# Autodesk Inventor assembly: Core
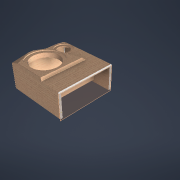
[picture p0: Inventor's stored thumbnail of the model, 180x180]
Saved by Autodesk Inventor 2022 (Build 260153000, 153)
## iProperties
Created: 2022-04-08
Part Number: Core
Document SubType Name: Assembly
Designer: Kalugin_a
Author: Kalugin_a
## Documents named in this file (9)
- D:\GitHUB\MELAS\Workspace\BoordyaBeatBox\Core.iam
- D:\GitHUB\MELAS\Workspace\BoordyaBeatBox\Front_L.ipt
- D:\GitHUB\MELAS\Workspace\BoordyaBeatBox\Front1.ipt
- Front1-hover.ipt
- D:\GitHUB\MELAS\Workspace\BoordyaBeatBox\Top.ipt
- D:\GitHUB\MELAS\Workspace\BoordyaBeatBox\side.ipt
- D:\GitHUB\MELAS\Workspace\BoordyaBeatBox\bottom.ipt
- D:\GitHUB\MELAS\Workspace\DIII\внутр.ipt
- D:\GitHUB\MELAS\Workspace\DIII\задник.ipt
## Components (8 placed, 7 different names)
1. Front_L:1 — Совмещение:1, Совмещение:2
2. Front1-hover:1
3. Top:1 — Совмещение:2, Совмещение:3, Совмещение:4
4. side:1 — Совмещение:1, Совмещение:3, Совмещение:5
5. bottom:1
6. side:2
7. внутр:1
8. задник:1 — Совмещение:4, Совмещение:5
## Relationships (5: Mate 5)
- Совмещение:1 [Mate]: Front_L:1 ↔ side:1
- Совмещение:2 [Mate]: Front_L:1 ↔ Top:1
- Совмещение:3 [Mate]: Top:1 ↔ side:1
- Совмещение:4 [Mate]: Top:1 ↔ задник:1
- Совмещение:5 [Mate]: side:1 ↔ задник:1
